# Autodesk Inventor assembly: Vizhutes-01-01-01
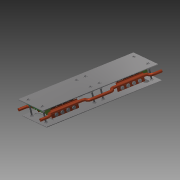
[picture p0: Inventor's stored thumbnail of the model, 180x180]
Saved by Autodesk Inventor 2015 SP1 (Build 190203100, 203)
## iProperties
Created: 2014-10-30
Part Number: Vizhutes-01-01-01
Document SubType Name: Assembly
Designer: laca
Author: laca
## Documents named in this file (10)
- C:\Users\laca\Desktop\RobotMechanikaForMAtlabVer2\VizhutesVer2.iam
- C:\Users\laca\Desktop\RobotMechanikaForMAtlabVer2\MotorVezerloHhid.iam
- C:\Users\laca\Desktop\RobotMechanikaForMAtlabVer2\NyakMotorVezerlo.ipt
- C:\Users\laca\Desktop\RobotMechanikaForMAtlabVer2\AlsoLemezVizhutesVer2.ipt
- C:\Users\laca\Desktop\RobotMechanikaForMAtlabVer2\FelsoLemezVizhutesVer2.ipt
- C:\Users\laca\Desktop\RobotMechanikaForMAtlabVer2\Alatet3csavarhoz.ipt
- C:\Users\laca\Desktop\RobotMechanikaForMAtlabVer2\3asAnya.ipt
- C:\Users\laca\Desktop\RobotMechanikaForMAtlabVer2\RezBorda.ipt
- C:\Users\laca\Desktop\RobotMechanikaForMAtlabVer2\Fi3es40mmcsavar.ipt
- C:\Users\laca\Desktop\RobotMechanikaForMAtlabVer2\Fi3es15mmcsavar.ipt
## Components (166 placed, 8 different names)
1. RezBorda:2 — Rotational:10, Rotational:17, Rotational:43, Rotational:45
2. RezBorda:1 — Rotational:7, Rotational:8, Rotational:16, Rotational:31, Rotational:35
3. MotorVezerloHhid:1 [sub-assembly] — Mate:1, Rotational:7, Rotational:17, Rotational:22, Rotational:23, Flush:4, Rotational:33, Rotational:46
4. MotorVezerloHhid:2 [sub-assembly] — Mate:1, Rotational:8, Rotational:10, Rotational:16, Rotational:37, Rotational:44
5. AlsoLemezVizhutesVer2:3 — Flush:4, Flush:5, Rotational:26, Rotational:27, Mate:2
6. FelsoLemezVizhutesVer2:2 — Flush:5, Rotational:28, Rotational:29, Mate:2
7. Fi3es15mmcsavar:1 — Rotational:32
8. Alatet3csavarhoz:42 — Rotational:31, Rotational:32
9. Alatet3csavarhoz:43 — Rotational:33, Rotational:34
10. 3asAnya:34 — Rotational:34
11. Fi3es15mmcsavar:2
12. Alatet3csavarhoz:44
13. Alatet3csavarhoz:45
14. 3asAnya:35
15. Fi3es15mmcsavar:3
16. Alatet3csavarhoz:46
17. Alatet3csavarhoz:47
18. 3asAnya:36
19. Fi3es15mmcsavar:4
20. Alatet3csavarhoz:48
21. Alatet3csavarhoz:49
22. 3asAnya:37
23. Fi3es15mmcsavar:5 — Rotational:36
24. Alatet3csavarhoz:51 — Rotational:35, Rotational:36
25. Alatet3csavarhoz:50 — Rotational:37, Rotational:38
26. 3asAnya:38 — Rotational:38
27. Fi3es15mmcsavar:7
28. Alatet3csavarhoz:52
29. Alatet3csavarhoz:53
30. 3asAnya:40
31. Fi3es15mmcsavar:8
32. Alatet3csavarhoz:54
33. Alatet3csavarhoz:55
34. 3asAnya:41
35. Fi3es15mmcsavar:9
36. Alatet3csavarhoz:56
37. Alatet3csavarhoz:57
38. 3asAnya:42
39. Fi3es15mmcsavar:10
40. Alatet3csavarhoz:58 — Rotational:46
41. 3asAnya:43
42. Alatet3csavarhoz:59 — Rotational:45
43. Fi3es15mmcsavar:12
44. Alatet3csavarhoz:62
45. 3asAnya:45
46. Alatet3csavarhoz:63
47. Fi3es15mmcsavar:13
48. Alatet3csavarhoz:64
49. 3asAnya:46
50. Alatet3csavarhoz:65
51. Fi3es15mmcsavar:14
52. Alatet3csavarhoz:66
53. 3asAnya:47
54. Alatet3csavarhoz:67
55. Fi3es15mmcsavar:11
56. Alatet3csavarhoz:60 — Rotational:44
57. 3asAnya:44
58. Alatet3csavarhoz:61 — Rotational:43
59. Fi3es15mmcsavar:15
60. Alatet3csavarhoz:68
61. 3asAnya:48
62. Alatet3csavarhoz:69
63. Fi3es15mmcsavar:16
64. Alatet3csavarhoz:70
65. 3asAnya:49
66. Alatet3csavarhoz:71
67. Fi3es15mmcsavar:17
68. Alatet3csavarhoz:72
69. 3asAnya:50
70. Alatet3csavarhoz:73
71. 3asAnya:5 — Rotational:30
72. Alatet3csavarhoz:6 — Rotational:29, Rotational:30
73. Fi3es40mmcsavar:1 — Rigid:1
74. 3asAnya:4 — Rotational:24, Insert:1
75. Alatet3csavarhoz:4 — Rotational:23, Rotational:24
76. 3asAnya:2 — Rotational:20, Rotational:21
77. 3asAnya:1 — Rotational:19, Rotational:20
78. Alatet3csavarhoz:2 — Rotational:19, Rotational:27
79. Alatet3csavarhoz:3 — Rotational:21, Rotational:22
80. Alatet3csavarhoz:1 — Rigid:1, Rotational:26
81. 3asAnya:3 — Insert:1, Rotational:25
82. Alatet3csavarhoz:5 — Rotational:25, Rotational:28
83. 3asAnya:6
84. Alatet3csavarhoz:7
85. Fi3es40mmcsavar:2
86. 3asAnya:7
87. Alatet3csavarhoz:8
88. 3asAnya:8
89. 3asAnya:9
90. Alatet3csavarhoz:9
91. Alatet3csavarhoz:10
92. Alatet3csavarhoz:11
93. 3asAnya:51
94. Alatet3csavarhoz:74
95. 3asAnya:10
96. Alatet3csavarhoz:12
97. Fi3es40mmcsavar:3
98. 3asAnya:11
99. Alatet3csavarhoz:13
100. 3asAnya:12
101. 3asAnya:13
102. Alatet3csavarhoz:14
103. Alatet3csavarhoz:15
104. Alatet3csavarhoz:16
105. 3asAnya:52
106. Alatet3csavarhoz:75
107. 3asAnya:14
108. Alatet3csavarhoz:17
109. Fi3es40mmcsavar:4
110. 3asAnya:15
111. Alatet3csavarhoz:18
112. 3asAnya:16
113. 3asAnya:17
114. Alatet3csavarhoz:19
115. Alatet3csavarhoz:20
116. Alatet3csavarhoz:21
117. 3asAnya:53
118. Alatet3csavarhoz:76
119. 3asAnya:18
120. Alatet3csavarhoz:22
121. Fi3es40mmcsavar:5
122. 3asAnya:19
123. Alatet3csavarhoz:23
124. 3asAnya:20
125. 3asAnya:21
126. Alatet3csavarhoz:24
127. Alatet3csavarhoz:25
128. Alatet3csavarhoz:26
129. 3asAnya:54
130. Alatet3csavarhoz:77
131. 3asAnya:22
132. Alatet3csavarhoz:27
133. Fi3es40mmcsavar:6
134. 3asAnya:23
135. Alatet3csavarhoz:28
136. 3asAnya:24
137. 3asAnya:25
138. Alatet3csavarhoz:29
139. Alatet3csavarhoz:30
140. Alatet3csavarhoz:31
141. 3asAnya:55
142. Alatet3csavarhoz:78
143. 3asAnya:26
144. Alatet3csavarhoz:32
145. Fi3es40mmcsavar:7
146. 3asAnya:27
147. Alatet3csavarhoz:33
148. 3asAnya:28
149. 3asAnya:29
150. Alatet3csavarhoz:34
151. Alatet3csavarhoz:35
152. Alatet3csavarhoz:36
153. 3asAnya:56
154. Alatet3csavarhoz:79
155. 3asAnya:30
156. Alatet3csavarhoz:37
157. Fi3es40mmcsavar:8
158. 3asAnya:31
159. Alatet3csavarhoz:38
160. 3asAnya:32
161. 3asAnya:33
162. Alatet3csavarhoz:39
163. Alatet3csavarhoz:40
164. Alatet3csavarhoz:41
165. 3asAnya:57
166. Alatet3csavarhoz:80
## Component patterns: (2 elements), (4 elements, first: Fi3es15mmcsavar:1 + Alatet3csavarhoz:42 + Alatet3csavarhoz:43 + 3asAnya:34), (4 elements, first: Fi3es15mmcsavar:5 + Alatet3csavarhoz:51 + Alatet3csavarhoz:50 + 3asAnya:38), (4 elements, first: Fi3es15mmcsavar:10 + Alatet3csavarhoz:58 + 3asAnya:43 + Alatet3csavarhoz:59), (4 elements, first: Fi3es15mmcsavar:11 + Alatet3csavarhoz:60 + 3asAnya:44 + Alatet3csavarhoz:61), (4 elements, first: 3asAnya:5 + Alatet3csavarhoz:6 + Fi3es40mmcsavar:1 + 3asAnya:4 + Alatet3csavarhoz:4 + 3asAnya:2 + 3asAnya:1 + Alatet3csavarhoz:2 + Alatet3csavarhoz:3 + Alatet3csavarhoz:1 + 3asAnya:3 + Alatet3csavarhoz:5), Component Pattern 8:2 (4 elements)
## Relationships (40: RevoluteJoint 33, Flush 3, Mate 2, WeldJoint 1, Insert 1)
- [Flush]: MotorVezerloHhid:1 ↔ MotorVezerloHhid:2
- Mate:1: MotorVezerloHhid:1 ↔ MotorVezerloHhid:2
- Rotational:7 [RevoluteJoint]: RezBorda:1 ↔ MotorVezerloHhid:1
- Rotational:8 [RevoluteJoint]: RezBorda:1 ↔ MotorVezerloHhid:2
- Rotational:10 [RevoluteJoint]: RezBorda:2 ↔ MotorVezerloHhid:2
- Rotational:16 [RevoluteJoint]: RezBorda:1 ↔ MotorVezerloHhid:2
- Rotational:17 [RevoluteJoint]: RezBorda:2 ↔ MotorVezerloHhid:1
- Rigid:1 [WeldJoint]: Fi3es40mmcsavar:1 ↔ Alatet3csavarhoz:1
- Rotational:19 [RevoluteJoint]: 3asAnya:1 ↔ Alatet3csavarhoz:2
- Rotational:20 [RevoluteJoint]: 3asAnya:2 ↔ 3asAnya:1
- Rotational:21 [RevoluteJoint]: 3asAnya:2 ↔ Alatet3csavarhoz:3
- Rotational:22 [RevoluteJoint]: MotorVezerloHhid:1 ↔ Alatet3csavarhoz:3
- Rotational:23 [RevoluteJoint]: MotorVezerloHhid:1 ↔ Alatet3csavarhoz:4
- Rotational:24 [RevoluteJoint]: 3asAnya:4 ↔ Alatet3csavarhoz:4
- Insert:1 (20 mm): 3asAnya:4 ↔ 3asAnya:3
- Rotational:25 [RevoluteJoint]: 3asAnya:3 ↔ Alatet3csavarhoz:5
- Flush:4: MotorVezerloHhid:1 ↔ AlsoLemezVizhutesVer2:3
- Flush:5: AlsoLemezVizhutesVer2:3 ↔ FelsoLemezVizhutesVer2:2
- Rotational:26 [RevoluteJoint]: AlsoLemezVizhutesVer2:3 ↔ Alatet3csavarhoz:1
- Rotational:27 [RevoluteJoint]: AlsoLemezVizhutesVer2:3 ↔ Alatet3csavarhoz:2
- Rotational:28 [RevoluteJoint]: FelsoLemezVizhutesVer2:2 ↔ Alatet3csavarhoz:5
- Rotational:29 [RevoluteJoint]: FelsoLemezVizhutesVer2:2 ↔ Alatet3csavarhoz:6
- Rotational:30 [RevoluteJoint]: 3asAnya:5 ↔ Alatet3csavarhoz:6
- Rotational:31 [RevoluteJoint]: RezBorda:1 ↔ Alatet3csavarhoz:42
- Rotational:32 [RevoluteJoint]: Fi3es15mmcsavar:1 ↔ Alatet3csavarhoz:42
- Rotational:33 [RevoluteJoint]: MotorVezerloHhid:1 ↔ Alatet3csavarhoz:43
- Rotational:34 [RevoluteJoint]: Alatet3csavarhoz:43 ↔ 3asAnya:34
- Rotational:35 [RevoluteJoint]: RezBorda:1 ↔ Alatet3csavarhoz:51
- Rotational:36 [RevoluteJoint]: Fi3es15mmcsavar:5 ↔ Alatet3csavarhoz:51
- Rotational:37 [RevoluteJoint]: MotorVezerloHhid:2 ↔ Alatet3csavarhoz:50
- Rotational:38 [RevoluteJoint]: Alatet3csavarhoz:50 ↔ 3asAnya:38
- [RevoluteJoint]: Fi3es15mmcsavar:10 ↔ Alatet3csavarhoz:59
- [RevoluteJoint]: Alatet3csavarhoz:58 ↔ 3asAnya:43
- [RevoluteJoint]: Fi3es15mmcsavar:11 ↔ Alatet3csavarhoz:61
- [RevoluteJoint]: Alatet3csavarhoz:60 ↔ 3asAnya:44
- Rotational:43 [RevoluteJoint]: RezBorda:2 ↔ Alatet3csavarhoz:61
- Rotational:44 [RevoluteJoint]: MotorVezerloHhid:2 ↔ Alatet3csavarhoz:60
- Rotational:45 [RevoluteJoint]: RezBorda:2 ↔ Alatet3csavarhoz:59
- Rotational:46 [RevoluteJoint]: MotorVezerloHhid:1 ↔ Alatet3csavarhoz:58
- Mate:2 (30 mm): AlsoLemezVizhutesVer2:3 ↔ FelsoLemezVizhutesVer2:2
## Named parameters: iTrigger0 = 2, JukaKoztiTavolsagHoszusag = 100 mm, JukakKoztiTavolsagSzeleseg = 53 mm, JukakANyakon = 3 mm, d57_1 = 12 mm, TranzisztoJukAtmero = 4 mm, d59_1 = 5 mm, d60_1 = 3 mm, d62_1 = 0 deg, d63_1 = 12 mm, d64_1 = 52 mm, d65_1 = 4 mm, d66_1 = 8 mm, d69_1 = 6 mm, d70_1 = 0 deg, TavolsagAKetNyakKozott = 18.167 mm, d212_d203 = -52.914296 deg, d213_d206 = 0 mm, d214_d207 = 26.713711 deg, d215_d202 = 0 mm, d216_d203 = -61.128244 deg, d217_d206 = 0 mm, d218_d207 = -147.994269 deg, d219_d202 = 0 mm
